# Autodesk Inventor assembly: roller cage
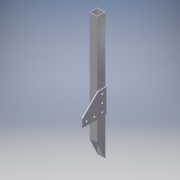
[picture p0: Inventor's stored thumbnail of the model, 180x180]
Saved by Autodesk Inventor 2016 (Build 200138000, 138)
## iProperties
Created: 2016-02-02
Part Number: roller cage
Document SubType Name: Assembly
Designer: gus
Mass: 119.442 g
Surface Area: 1363.6 cm^2
Volume: 119.442 cm^3
Density: 1 g/cm^3
Author: gus
## Documents named in this file (3)
- \\Mac\Home\Desktop\1510-stronghold-CAD-master\roller cage\roller cage.iam
- \\Mac\Home\Desktop\1510-stronghold-CAD-master\roller cage\top.ipt
- \\Mac\Home\Desktop\1510-stronghold-CAD-master\roller cage\gusset plate.ipt
## Components (2 placed, 2 different names)
1. top:1 — Flush:5, Mate:3
2. gusset plate:2 — Flush:5, Mate:3
## Relationships (2: Flush 1, Mate 1)
- Flush:5: top:1 ↔ gusset plate:2
- Mate:3: top:1 ↔ gusset plate:2
